# Autodesk Inventor assembly: bogie_right
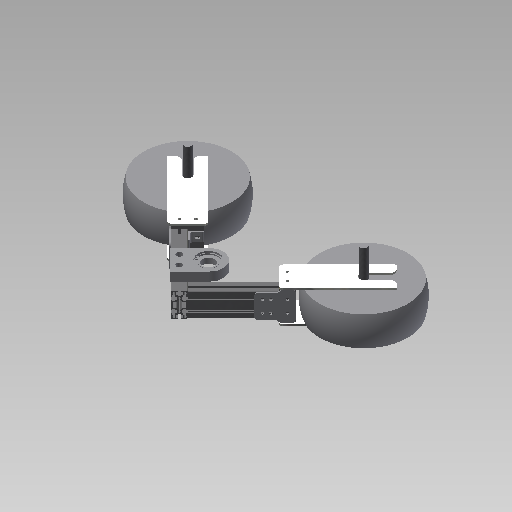
[picture p0: Inventor's stored thumbnail of the model, 512x512]
Saved by Autodesk Inventor 2021.2 (Build 252289000, 289)
## iProperties
Created: 2021-05-27
Part Number: bogie_right
Document SubType Name: Assembly
Designer: gisen
Author: gisen
## Documents named in this file (7)
- C:\Users\gisen\workspace\beetle_inventor_model\suspension\bogie_right.iam
- C:\Users\gisen\workspace\beetle_inventor_model\suspension\AFS-2040-4-130_right.ipt
- C:\Users\gisen\workspace\beetle_inventor_model\suspension\AFS-2040-4-110_right.ipt
- C:\Users\gisen\workspace\beetle_inventor_model\suspension\SBGSMA6904ZZ-35\SBGSMA6904ZZ-35_right.iam
- C:\Users\gisen\workspace\beetle_inventor_model\suspension\wheel_with_mounts_right.iam
- C:\Users\gisen\workspace\beetle_inventor_model\suspension\M4L_right.ipt
- C:\Users\gisen\workspace\beetle_inventor_model\suspension\wheel_frame_mount_right.ipt
## Components (8 placed, 3 different names)
1. Part1:1 — フラッシュ:14, フラッシュ:2, フラッシュ:1, メイト:1, 対称度:1, メイト:6, メイト:5, 角度:1, フラッシュ:20, メイト:21, メイト:19
2. Part1:2 — フラッシュ:2, フラッシュ:1, メイト:1, 対称度:1, メイト:24, メイト:22
3. SBGSMA6904ZZ-35_right:1 [sub-assembly] — メイト:7, メイト:6, メイト:5, 角度:1
4. wheel_with_mounts_right:1 [sub-assembly] — フラッシュ:19, メイト:18, メイト:17, フラッシュ:18, 対称度:2, メイト:25, メイト:23
5. wheel_with_mounts_right:2 [sub-assembly] — フラッシュ:20, メイト:17, フラッシュ:18, メイト:15, 対称度:2, メイト:20, フラッシュ:21
6. Part1:3 — メイト:21, メイト:20, メイト:19
7. Part1:4 — フラッシュ:21
8. Part1:5 — メイト:25, メイト:24, メイト:23, メイト:22
## Relationships (24: Mate 15, Flush 6, Symmetry 2, Angle 1)
- フラッシュ:14 [Flush]: Part1:1
- フラッシュ:2 [Flush]: Part1:1 ↔ Part1:2
- フラッシュ:1 [Flush]: Part1:1 ↔ Part1:2
- メイト:1 [Mate]: Part1:1 ↔ Part1:2
- 対称度:1 [Symmetry]: Part1:1 ↔ Part1:2
- メイト:7 [Mate]: SBGSMA6904ZZ-35_right:1
- メイト:6 [Mate]: Part1:1 ↔ SBGSMA6904ZZ-35_right:1
- メイト:5 [Mate]: Part1:1 ↔ SBGSMA6904ZZ-35_right:1
- 角度:1 [Angle] (0 deg): Part1:1 ↔ SBGSMA6904ZZ-35_right:1
- フラッシュ:19 [Flush]: wheel_with_mounts_right:1
- メイト:18 [Mate]: wheel_with_mounts_right:1
- フラッシュ:20 [Flush]: Part1:1 ↔ wheel_with_mounts_right:2
- メイト:17 [Mate] (300 mm): wheel_with_mounts_right:1 ↔ wheel_with_mounts_right:2
- フラッシュ:18 [Flush]: wheel_with_mounts_right:1 ↔ wheel_with_mounts_right:2
- メイト:15 [Mate]: wheel_with_mounts_right:2
- 対称度:2 [Symmetry]: wheel_with_mounts_right:1 ↔ wheel_with_mounts_right:2
- メイト:21 [Mate] (-10 mm): Part1:1 ↔ Part1:3
- メイト:20 [Mate]: wheel_with_mounts_right:2 ↔ Part1:3
- メイト:19 [Mate]: Part1:1 ↔ Part1:3
- フラッシュ:21 [Mate]: wheel_with_mounts_right:2 ↔ Part1:4
- メイト:25 [Mate] (-10 mm): wheel_with_mounts_right:1 ↔ Part1:5
- メイト:24 [Mate] (-10 mm): Part1:2 ↔ Part1:5
- メイト:23 [Mate] (-10 mm): wheel_with_mounts_right:1 ↔ Part1:5
- メイト:22 [Mate]: Part1:2 ↔ Part1:5
